# Autodesk Inventor assembly: Drivetrain Side
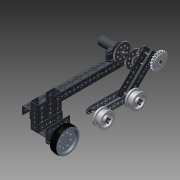
[picture p0: Inventor's stored thumbnail of the model, 180x180]
Saved by Autodesk Inventor 2015 (Build 190159000, 159)
## iProperties
Created: 2015-09-28
Part Number: Drivetrain Side
Document SubType Name: Assembly
Designer: Jing-Chen
Author: Jing-Chen
## Documents named in this file (14)
- C:\Users\Jing-Chen\Desktop\Bionic Hybrids 2016\Bionic-Hybrids\CAD\Drivetrain\Sub-Assemblies\Drivetrain Side.iam
- C:\Users\Jing-Chen\Desktop\Bionic Hybrids 2016\Bionic-Hybrids\Stock\Bracket-U25 - 739069.ipt
- C:\Users\Jing-Chen\Desktop\Bionic Hybrids 2016\Bionic-Hybrids\CAD\Drivetrain\Sub-Assemblies\Wheel Assembly.iam
- C:\Users\Jing-Chen\Desktop\Bionic Hybrids 2016\Bionic-Hybrids\CAD\Drivetrain\Sub-Assemblies\Track Frame Assembly.iam
- C:\Users\Jing-Chen\Desktop\Bionic Hybrids 2016\Bionic-Hybrids\Stock\Bearing-Thrust - 739091.ipt
- C:\Users\Jing-Chen\Desktop\Bionic Hybrids 2016\Bionic-Hybrids\Stock\Motor Mount - 739089.ipt
- C:\Users\Jing-Chen\Desktop\Bionic Hybrids 2016\Bionic-Hybrids\Stock\Bracket-U5 - 739066.ipt
- C:\Users\Jing-Chen\Desktop\Bionic Hybrids 2016\Bionic-Hybrids\CAD\Drivetrain\Modified Parts\Movable Motor.iam
- C:\Users\Jing-Chen\Desktop\Bionic Hybrids 2016\Bionic-Hybrids\Stock\Sample Worm Gear Assembly.iam
- C:\Users\Jing-Chen\Desktop\Bionic Hybrids 2016\Bionic-Hybrids\Stock\Shaft Coupler-4.75mm - 739275.iam
- C:\Users\Jing-Chen\Desktop\Bionic Hybrids 2016\Bionic-Hybrids\Stock\Gear-80 tooth - 731901.ipt
- C:\Users\Jing-Chen\Desktop\Bionic Hybrids 2016\Bionic-Hybrids\Stock\Plate-2x1 Long - 739061.ipt
- C:\Users\Jing-Chen\Desktop\Bionic Hybrids 2016\Bionic-Hybrids\Stock\Shaft Collar-Setscrew, Axle, Mountable - 739079.iam
- C:\Users\Jing-Chen\Desktop\Bionic Hybrids 2016\Bionic-Hybrids\Stock\Screw 0.5in - 739097.ipt
## Components (21 placed, 13 different names)
1. Track Frame Assembly:1 [sub-assembly] — Mate:33, Mate:36, Rotation:1, Flush:4
2. Bearing-Thrust - 739091:1 — Mate:33, Mate:36, Mate:60, Mate:61
3. Motor Mount - 739089:1 — Mate:40, Flush:1, Mate:51, Mate:52, Mate:53
4. Wheel Assembly:1 [sub-assembly] — Angle:2, Mate:41, Flush:2
5. Movable Motor:1 [sub-assembly] — Mate:40, Flush:1, Angle:1, Angle:2, Mate:41, Flush:2
6. Bracket-U5 - 739066:1 — Mate:44, Mate:46, Mate:47, Mate:51, Mate:52, Mate:53
7. Bracket-U5 - 739066:2 — Mate:44, Mate:46, Mate:47, Mate:54, Mate:55, Mate:56
8. Bracket-U5 - 739066:3 — Mate:57, Mate:58, Mate:59
9. Sample Worm Gear Assembly:2 [sub-assembly]
10. Shaft Coupler-4.75mm - 739275:1 [sub-assembly]
11. Bracket-U25 - 739069:1 — Mate:54, Mate:55, Mate:56, Mate:57, Mate:58, Mate:59, Mate:60, Mate:61, Mate:62, Angle:3, Mate:81
12. Movable Motor:2 [sub-assembly] — Mate:64, Flush:3, Angle:4, Mate:80, Angle:5
13. Motor Mount - 739089:2 — Mate:62, Angle:3, Mate:64, Flush:3, Mate:76, Mate:77, Mate:78, Mate:82, Mate:83
14. Gear-80 tooth - 731901:1 — Mate:80, Rotation:1, Flush:4, Mate:85, Mate:86, Mate:87, Mate:88, Mate:89, Mate:90, Mate:91, Mate:92, Mate:93, Mate:94, Mate:95
15. Plate-2x1 Long - 739061:1 — Mate:76, Mate:77, Mate:78, Mate:84
16. Plate-2x1 Long - 739061:2 — Mate:81, Mate:82, Mate:83, Mate:84
17. Shaft Collar-Setscrew, Axle, Mountable - 739079:1 [sub-assembly] — Mate:85, Angle:5, Mate:86, Mate:87
18. Screw 0.5in - 739097:1 — Mate:91, Mate:92
19. Screw 0.5in - 739097:2 — Mate:90, Mate:93
20. Screw 0.5in - 739097:3 — Mate:88, Mate:95
21. Screw 0.5in - 739097:4 — Mate:89, Mate:94
## Relationships (49: Mate 39, Angle 5, Flush 4, RelateRotation 1)
- Mate:33: Track Frame Assembly:1 ↔ Bearing-Thrust - 739091:1
- Mate:36: Track Frame Assembly:1 ↔ Bearing-Thrust - 739091:1
- Mate:40: Motor Mount - 739089:1 ↔ Movable Motor:1
- Flush:1: Motor Mount - 739089:1 ↔ Movable Motor:1
- Angle:1 (180 deg): Movable Motor:1
- Angle:2 (180 deg): Wheel Assembly:1 ↔ Movable Motor:1
- Mate:41: Wheel Assembly:1 ↔ Movable Motor:1
- Flush:2: Wheel Assembly:1 ↔ Movable Motor:1
- Mate:44: Bracket-U5 - 739066:1 ↔ Bracket-U5 - 739066:2
- Mate:46: Bracket-U5 - 739066:1 ↔ Bracket-U5 - 739066:2
- Mate:47: Bracket-U5 - 739066:1 ↔ Bracket-U5 - 739066:2
- Mate:51: Motor Mount - 739089:1 ↔ Bracket-U5 - 739066:1
- Mate:52: Motor Mount - 739089:1 ↔ Bracket-U5 - 739066:1
- Mate:53: Motor Mount - 739089:1 ↔ Bracket-U5 - 739066:1
- Mate:54: Bracket-U5 - 739066:2 ↔ Bracket-U25 - 739069:1
- Mate:55: Bracket-U5 - 739066:2 ↔ Bracket-U25 - 739069:1
- Mate:56: Bracket-U5 - 739066:2 ↔ Bracket-U25 - 739069:1
- Mate:57: Bracket-U5 - 739066:3 ↔ Bracket-U25 - 739069:1
- Mate:58: Bracket-U5 - 739066:3 ↔ Bracket-U25 - 739069:1
- Mate:59: Bracket-U5 - 739066:3 ↔ Bracket-U25 - 739069:1
- Mate:60: Bearing-Thrust - 739091:1 ↔ Bracket-U25 - 739069:1
- Mate:61: Bearing-Thrust - 739091:1 ↔ Bracket-U25 - 739069:1
- Mate:62: Bracket-U25 - 739069:1 ↔ Motor Mount - 739089:2
- Angle:3 (0 deg): Bracket-U25 - 739069:1 ↔ Motor Mount - 739089:2
- Mate:64: Movable Motor:2 ↔ Motor Mount - 739089:2
- Flush:3: Movable Motor:2 ↔ Motor Mount - 739089:2
- Angle:4 (135 deg): Movable Motor:2
- Mate:76: Motor Mount - 739089:2 ↔ Plate-2x1 Long - 739061:1
- Mate:77: Motor Mount - 739089:2 ↔ Plate-2x1 Long - 739061:1
- Mate:78: Motor Mount - 739089:2 ↔ Plate-2x1 Long - 739061:1
- Mate:80: Movable Motor:2 ↔ Gear-80 tooth - 731901:1
- Mate:81: Bracket-U25 - 739069:1 ↔ Plate-2x1 Long - 739061:2
- Mate:82: Motor Mount - 739089:2 ↔ Plate-2x1 Long - 739061:2
- Mate:83: Motor Mount - 739089:2 ↔ Plate-2x1 Long - 739061:2
- Mate:84: Plate-2x1 Long - 739061:1 ↔ Plate-2x1 Long - 739061:2
- Rotation:1 [RelateRotation] (1 ul): Track Frame Assembly:1 ↔ Gear-80 tooth - 731901:1
- Flush:4: Track Frame Assembly:1 ↔ Gear-80 tooth - 731901:1
- Mate:85: Gear-80 tooth - 731901:1 ↔ Shaft Collar-Setscrew, Axle, Mountable - 739079:1
- Angle:5 (180 deg): Movable Motor:2 ↔ Shaft Collar-Setscrew, Axle, Mountable - 739079:1
- Mate:86: Gear-80 tooth - 731901:1 ↔ Shaft Collar-Setscrew, Axle, Mountable - 739079:1
- Mate:87: Gear-80 tooth - 731901:1 ↔ Shaft Collar-Setscrew, Axle, Mountable - 739079:1
- Mate:88: Gear-80 tooth - 731901:1 ↔ Screw 0.5in - 739097:3
- Mate:89: Gear-80 tooth - 731901:1 ↔ Screw 0.5in - 739097:4
- Mate:90: Gear-80 tooth - 731901:1 ↔ Screw 0.5in - 739097:2
- Mate:91: Gear-80 tooth - 731901:1 ↔ Screw 0.5in - 739097:1
- Mate:92: Gear-80 tooth - 731901:1 ↔ Screw 0.5in - 739097:1
- Mate:93: Gear-80 tooth - 731901:1 ↔ Screw 0.5in - 739097:2
- Mate:94: Gear-80 tooth - 731901:1 ↔ Screw 0.5in - 739097:4
- Mate:95: Gear-80 tooth - 731901:1 ↔ Screw 0.5in - 739097:3
